# Autodesk Inventor assembly: CompleteAssembly
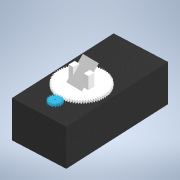
[picture p0: Inventor's stored thumbnail of the model, 180x180]
Saved by Autodesk Inventor 2022.2 (Build 262287010, 287A)
## iProperties
Created: 2022-05-02
Part Number: CompleteAssembly
Document SubType Name: Assembly
Designer: mabel
Author: mabel
## Documents named in this file (14)
- D:\GitHub\laser-nav\Mechanics\Final Prototype\CompleteAssembly.iam
- C:\Users\mabel\OneDrive\Documentos\Inventor\LaserNavigationSystem\Mecanizado\TapaconEjeM.ipt
- C:\Users\mabel\OneDrive\Documentos\Inventor\LaserNavigationSystem\Cambio\EngraneN18.ipt
- C:\Users\mabel\OneDrive\Documentos\Inventor\LaserNavigationSystem\Cambio\EngraneN72.ipt
- C:\Users\mabel\OneDrive\Documentos\Inventor\LaserNavigationSystem\Mecanizado\Caja.ipt
- C:\Users\mabel\OneDrive\Documentos\Inventor\LaserNavigationSystem\Pruebas-ultimo\Base.ipt
- C:\Users\mabel\OneDrive\Documentos\Inventor\LaserNavigationSystem\Pruebas-ultimo\BaseL.ipt
- C:\Users\mabel\OneDrive\Documentos\Inventor\LaserNavigationSystem\SoporteDerecho.ipt
- C:\Users\mabel\OneDrive\Documentos\Inventor\LaserNavigationSystem\SoporteIzquierdo.ipt
- C:\Users\mabel\OneDrive\Documentos\Inventor\LaserNavigationSystem\BeamSplitter.ipt
- C:\Users\mabel\OneDrive\Documentos\Inventor\LaserNavigationSystem\Cambio\SoportaEspejo.ipt
- C:\Users\mabel\OneDrive\Documentos\Inventor\LaserNavigationSystem\SoporteLente.ipt
- C:\Users\mabel\OneDrive\Documentos\Inventor\LaserNavigationSystem\SoporteSensor.ipt
- C:\Users\mabel\OneDrive\Documentos\Inventor\LaserNavigationSystem\Lente.ipt
## Components (13 placed, 13 different names)
1. Engranaje rectoN18:1 — Coincidencia:3, Coincidencia:22
2. Engranaje rectoN72:1 — Coincidencia:1, Coincidencia:2, Coincidencia:10, Coincidencia:11, Coincidencia:23, Coincidencia:24
3. TapaconEjeM:1 — Coincidencia:1, Coincidencia:2, Coincidencia:3, Nivelación:1, Nivelación:2, Coincidencia:22
4. Caja:1 — Nivelación:1, Nivelación:2, Coincidencia:4, Coincidencia:5, Coincidencia:6, Coincidencia:7, Coincidencia:8, Coincidencia:9, Coincidencia:17, Coincidencia:18, Coincidencia:19, Coincidencia:20, Coincidencia:21
5. Base:1 — Coincidencia:4, Coincidencia:5, Coincidencia:6, Coincidencia:12
6. BaseL:1 — Coincidencia:7, Coincidencia:8, Coincidencia:9, Coincidencia:13
7. SoporteDerecho:1 — Coincidencia:10
8. SoporteIzquierdo:1 — Coincidencia:11
9. BeamSplitter:1 — Coincidencia:12, Coincidencia:13
10. SoportaEspejo:1 — Coincidencia:23, Coincidencia:24
11. SoporteLente:1 — Coincidencia:17, Coincidencia:18, Insertar:1
12. SoporteSensor:1 — Coincidencia:19, Coincidencia:20, Coincidencia:21
13. Lente:1 — Insertar:1
## Relationships (24: Mate 21, Flush 2, Insert 1)
- Coincidencia:1 [Mate]: Engranaje rectoN72:1 ↔ TapaconEjeM:1
- Coincidencia:2 [Mate]: Engranaje rectoN72:1 ↔ TapaconEjeM:1
- Coincidencia:3 [Mate]: Engranaje rectoN18:1 ↔ TapaconEjeM:1
- Nivelación:1 [Flush]: TapaconEjeM:1 ↔ Caja:1
- Nivelación:2 [Flush]: TapaconEjeM:1 ↔ Caja:1
- Coincidencia:4 [Mate]: Caja:1 ↔ Base:1
- Coincidencia:5 [Mate]: Caja:1 ↔ Base:1
- Coincidencia:6 [Mate]: Caja:1 ↔ Base:1
- Coincidencia:7 [Mate]: Caja:1 ↔ BaseL:1
- Coincidencia:8 [Mate]: Caja:1 ↔ BaseL:1
- Coincidencia:9 [Mate]: Caja:1 ↔ BaseL:1
- Coincidencia:10 [Mate]: Engranaje rectoN72:1 ↔ SoporteDerecho:1
- Coincidencia:11 [Mate]: Engranaje rectoN72:1 ↔ SoporteIzquierdo:1
- Coincidencia:12 [Mate]: Base:1 ↔ BeamSplitter:1
- Coincidencia:13 [Mate]: BaseL:1 ↔ BeamSplitter:1
- Coincidencia:17 [Mate]: Caja:1 ↔ SoporteLente:1
- Coincidencia:18 [Mate] (100 mm): Caja:1 ↔ SoporteLente:1
- Coincidencia:19 [Mate]: Caja:1 ↔ SoporteSensor:1
- Coincidencia:20 [Mate]: Caja:1 ↔ SoporteSensor:1
- Coincidencia:21 [Mate]: Caja:1 ↔ SoporteSensor:1
- Insertar:1: SoporteLente:1 ↔ Lente:1
- Coincidencia:22 [Mate]: Engranaje rectoN18:1 ↔ TapaconEjeM:1
- Coincidencia:23 [Mate]: Engranaje rectoN72:1 ↔ SoportaEspejo:1
- Coincidencia:24 [Mate]: Engranaje rectoN72:1 ↔ SoportaEspejo:1
